# Autodesk Inventor assembly: ASY MSC 900.1 base frame
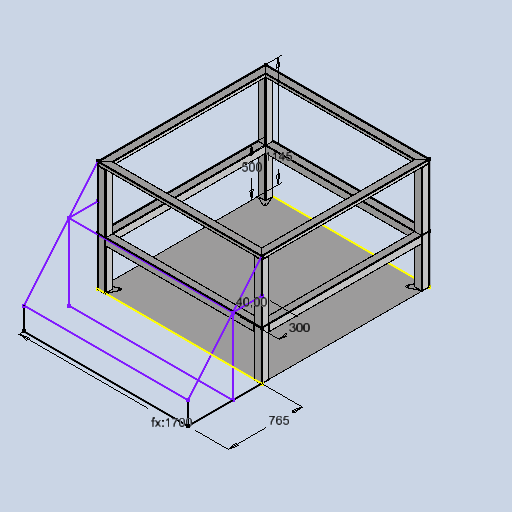
[picture p0: Inventor's stored thumbnail of the model, 512x512]
Saved by Autodesk Inventor 2025 (Build 290162010, 162A)
## iProperties
Created: 2024-05-19
Part Number: ASY MSC 900.1 base frame
Document SubType Name: Assembly
Designer: admin
Stock Number: ASY МОО 900.1 рама основания
_SolveAssemblyDoc: Frame Generator Solve Assembly
_Version: 15.0.0
Author: admin
## Documents named in this file (4)
- C:\Users\pokla\Documents\Inventor\Manturovo2\ASY MSC 900.1 base frame.iam
- C:\Users\pokla\Documents\Inventor\Manturovo2\MSC DIM 009.1 base frame sketch.ipt
- C:\Users\pokla\Documents\Inventor\Manturovo2\Pillars\ASY MSC 900.1.1 base frame.iam
- C:\Users\pokla\Documents\Inventor\Manturovo2\MSC 128 base plate.ipt
## Components (6 placed, 3 different names)
1. MSC DIM 009.1 base frame sketch.ipt:1
2. ASY MSC 900.1.1 base frame.iam:1 [sub-assembly] — Rigid:1, Rigid:2, Rigid:3, Rigid:4
3. MSC 128 base plate.ipt:1 — Rigid:2
4. MSC 128 base plate.ipt:2 — Rigid:1
5. MSC 128 base plate.ipt:3 — Rigid:4
6. MSC 128 base plate.ipt:4 — Rigid:3
## Relationships (4: WeldJoint 4)
- Rigid:1 [WeldJoint]: ASY MSC 900.1.1 base frame.iam:1 ↔ MSC 128 base plate.ipt:2
- Rigid:2 [WeldJoint]: ASY MSC 900.1.1 base frame.iam:1 ↔ MSC 128 base plate.ipt:1
- Rigid:3 [WeldJoint]: ASY MSC 900.1.1 base frame.iam:1 ↔ MSC 128 base plate.ipt:4
- Rigid:4 [WeldJoint]: ASY MSC 900.1.1 base frame.iam:1 ↔ MSC 128 base plate.ipt:3
